# Autodesk Inventor assembly: SubAssembly Undercarriage
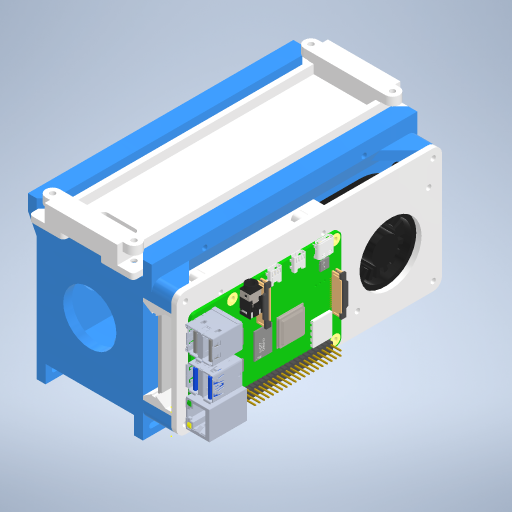
[picture p0: Inventor's stored thumbnail of the model, 512x512]
Saved by Autodesk Inventor 2023 (Build 270158000, 158)
## iProperties
Created: 2023-01-18
Part Number: SubAssembly Undercarriage
Document SubType Name: Assembly
Designer: Administrator
Author: Administrator
## Documents named in this file (7)
- D:\Documents\GitHub\WU-Team20-AutonomousDrone\CAD\ASSEMBLY\SubAssembly - BatteryCarrier WithAccessories.iam
- D:\Documents\GitHub\WU-Team20-AutonomousDrone\CAD\Electronics Mounts\BatteryCarrier - SlidingPlate Main.ipt
- D:\Documents\GitHub\WU-Team20-AutonomousDrone\CAD\Raw Models\BlowerFan.ipt
- D:\Documents\GitHub\WU-Team20-AutonomousDrone\CAD\Electronics Mounts\BatteryCarrier - SlidingPlate ToothedMount.ipt
- D:\Documents\GitHub\WU-Team20-AutonomousDrone\CAD\Raw Models\Raspberry Pi Model 4B\Raspberry Pi 4 Model B.iam
- D:\Documents\GitHub\WU-Team20-AutonomousDrone\CAD\Electronics Mounts\ChargingCircuit - ShroudPlate - Version2.ipt
- D:\Documents\GitHub\WU-Team20-AutonomousDrone\CAD\Raw Models\BQ24600 PCB Mockup.ipt
## Components (6 placed, 6 different names)
1. BatteryCarrier - SlidingPlate Main:1 — Mate:3, Flush:1, Mate:4
2. BlowerFan:1
3. ChargingCircuit - ShroudPlate - Version2:1 — Mate:5, Mate:6
4. BatteryCarrier - SlidingPlate ToothedMount:1 — Mate:3, Flush:1, Mate:4
5. Raspberry Pi 4 Model B:1 [sub-assembly]
6. BQ24600 PCB Mockup:1 — Mate:5, Mate:6
## Relationships (9: Mate 6, WeldJoint 2, Flush 1)
- [Mate]: BlowerFan:1 ↔ ChargingCircuit - ShroudPlate - Version2:1
- [Mate]: BlowerFan:1 ↔ ChargingCircuit - ShroudPlate - Version2:1
- [WeldJoint]: BatteryCarrier - SlidingPlate Main:1 ↔ ChargingCircuit - ShroudPlate - Version2:1
- Mate:3 (0.25 mm): BatteryCarrier - SlidingPlate Main:1 ↔ BatteryCarrier - SlidingPlate ToothedMount:1
- Flush:1 (-5 mm): BatteryCarrier - SlidingPlate Main:1 ↔ BatteryCarrier - SlidingPlate ToothedMount:1
- Mate:4 (0.5 mm): BatteryCarrier - SlidingPlate Main:1 ↔ BatteryCarrier - SlidingPlate ToothedMount:1
- [WeldJoint] (5 mm): ChargingCircuit - ShroudPlate - Version2:1 ↔ Raspberry Pi 4 Model B:1
- Mate:5: ChargingCircuit - ShroudPlate - Version2:1 ↔ BQ24600 PCB Mockup:1
- Mate:6: ChargingCircuit - ShroudPlate - Version2:1 ↔ BQ24600 PCB Mockup:1
